# Autodesk Inventor assembly: Button_red
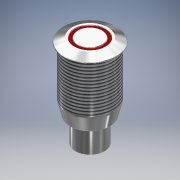
[picture p0: Inventor's stored thumbnail of the model, 180x180]
Saved by Autodesk Inventor 2016 (Build 200138000, 138)
## iProperties
Created: 2016-04-10
Part Number: Button_red
Document SubType Name: Assembly
Designer: agmle
Author: agmle
## Documents named in this file (3)
- C:\Users\agmle\BitTorrent Sync\private\projects\Creekfleet_Timer\hardware\CAD\Main\Button_red.iam
- C:\Users\agmle\BitTorrent Sync\private\projects\Creekfleet_Timer\hardware\CAD\Main\Button_housing.ipt
- C:\Users\agmle\BitTorrent Sync\private\projects\Creekfleet_Timer\hardware\CAD\Main\Button_ring.ipt
## Components (2 placed, 2 different names)
1. Button_housing:1 — Insert:1
2. Button_ring:1 — Insert:1
## Relationships (1: Insert 1)
- Insert:1: Button_housing:1 ↔ Button_ring:1
